# Autodesk Inventor assembly: BasicAssembly
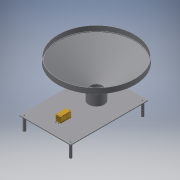
[picture p0: Inventor's stored thumbnail of the model, 180x180]
Saved by Autodesk Inventor 2019 (Build 230136000, 136)
## iProperties
Created: 2018-12-14
Part Number: BasicAssembly
Document SubType Name: Assembly
Designer: jmc
Author: jmc
## Documents named in this file (6)
- C:\Users\l0086\Desktop\CatFeeder\BasicAssembly.iam
- C:\Users\l0086\Desktop\CatFeeder\Cono.ipt
- C:\Users\l0086\Desktop\CatFeeder\BaseDelCono.ipt
- C:\Users\l0086\Desktop\CatFeeder\ServoHitecD930.ipt
- C:\Users\l0086\Desktop\CatFeeder\Base.ipt
- C:\Users\l0086\Desktop\CatFeeder\Trampilla.ipt
## Components (5 placed, 5 different names)
1. Cono:1 — Rigid:1
2. BaseDelCono:1 — Rigid:1, Rigid:2, Rigid:3, Angle:1
3. ServoHitecD930:1 — Rigid:2
4. Base:1 — Rigid:3
5. Trampilla:1 — Mate:1
## Relationships (5: WeldJoint 3, Mate 1, Angle 1)
- Rigid:1 [WeldJoint]: Cono:1 ↔ BaseDelCono:1
- Rigid:2 [WeldJoint]: BaseDelCono:1 ↔ ServoHitecD930:1
- Rigid:3 [WeldJoint]: BaseDelCono:1 ↔ Base:1
- Mate:1: Trampilla:1
- Angle:1 (90 deg): BaseDelCono:1
